# Autodesk Inventor assembly: Cabeza
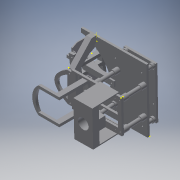
[picture p0: Inventor's stored thumbnail of the model, 180x180]
Saved by Autodesk Inventor 2017 SP1 (Build 210196100, 196)
## iProperties
Part Number: Cabeza
Material: Genérico
Document SubType Name: Assembly
Designer: Juan
Author: Juan
## Documents named in this file (13)
- C:\Users\Juan\Documents\Inventor\Cabeza_1\Cabeza.iam
- C:\Users\Juan\Documents\Inventor\Cabeza_1\BaseSuperior.ipt
- C:\Users\Juan\Documents\Inventor\Cabeza_1\Base.ipt
- C:\Users\Juan\Documents\Inventor\Cabeza_1\PosteLargo.ipt
- C:\Users\Juan\Documents\Inventor\Cabeza_1\PosteV.ipt
- C:\Users\Juan\Documents\Inventor\Cabeza_1\PosteCorto.ipt
- C:\Users\Juan\Documents\Inventor\Cabeza_1\BaseRB.ipt
- C:\Users\Juan\Documents\Inventor\Cabeza_1\SoporteCuello.ipt
- C:\Users\Juan\Documents\Inventor\Cabeza_1\PuenteMandibula.ipt
- C:\Users\Juan\Documents\Inventor\Cabeza_1\Mandibula.ipt
- C:\Users\Juan\Documents\Inventor\Cabeza_1\Puente.ipt
- C:\Users\Juan\Documents\Inventor\Cabeza_1\SoporteOjos.ipt
- C:\Users\Juan\Documents\Inventor\Cabeza_1\ojo.ipt
## Components (19 placed, 12 different names)
1. BaseSuperior:1 — Coincidencia:2, Coincidencia:3, Coincidencia:4, Coincidencia:5, Coincidencia:11, Coincidencia:14, Coincidencia:19
2. Base:1 — Coincidencia:7, Coincidencia:8, Coincidencia:9, Coincidencia:10, Coincidencia:12, Coincidencia:13, Coincidencia:15, Coincidencia:16, Coincidencia:17
3. PosteCorto:2 — Coincidencia:5
4. PosteCorto:3 — Coincidencia:4
5. PosteCorto:4 — Coincidencia:2
6. PosteCorto:5 — Coincidencia:3, Coincidencia:6
7. BaseRB:1 — Coincidencia:6
8. PosteLargo:2 — Coincidencia:9
9. PosteLargo:3 — Coincidencia:10, Coincidencia:14
10. PosteLargo:4 — Coincidencia:8
11. PosteLargo:5 — Coincidencia:7, Coincidencia:11
12. PosteV:1 — Coincidencia:12, Coincidencia:13
13. SoporteCuello:1 — Coincidencia:15, Coincidencia:16
14. PuenteMandibula:1 — Coincidencia:17, Coincidencia:18
15. Mandibula:1 — Coincidencia:18
16. Puente:1 — Coincidencia:19, Coincidencia:20
17. SoporteOjos:1 — Coincidencia:20, Coincidencia:21, Coincidencia:22
18. ojo:1 — Coincidencia:21
19. ojo:2 — Coincidencia:22
## Relationships (21: Mate 21)
- Coincidencia:2 [Mate]: BaseSuperior:1 ↔ PosteCorto:4
- Coincidencia:3 [Mate]: BaseSuperior:1 ↔ PosteCorto:5
- Coincidencia:4 [Mate]: BaseSuperior:1 ↔ PosteCorto:3
- Coincidencia:5 [Mate]: BaseSuperior:1 ↔ PosteCorto:2
- Coincidencia:6 [Mate]: PosteCorto:5 ↔ BaseRB:1
- Coincidencia:7 [Mate]: Base:1 ↔ PosteLargo:5
- Coincidencia:8 [Mate]: Base:1 ↔ PosteLargo:4
- Coincidencia:9 [Mate]: Base:1 ↔ PosteLargo:2
- Coincidencia:10 [Mate]: Base:1 ↔ PosteLargo:3
- Coincidencia:11 [Mate]: BaseSuperior:1 ↔ PosteLargo:5
- Coincidencia:12 [Mate]: Base:1 ↔ PosteV:1
- Coincidencia:13 [Mate]: Base:1 ↔ PosteV:1
- Coincidencia:14 [Mate]: BaseSuperior:1 ↔ PosteLargo:3
- Coincidencia:15 [Mate]: Base:1 ↔ SoporteCuello:1
- Coincidencia:16 [Mate]: Base:1 ↔ SoporteCuello:1
- Coincidencia:17 [Mate]: Base:1 ↔ PuenteMandibula:1
- Coincidencia:18 [Mate]: PuenteMandibula:1 ↔ Mandibula:1
- Coincidencia:19 [Mate]: BaseSuperior:1 ↔ Puente:1
- Coincidencia:20 [Mate]: Puente:1 ↔ SoporteOjos:1
- Coincidencia:21 [Mate]: SoporteOjos:1 ↔ ojo:1
- Coincidencia:22 [Mate]: SoporteOjos:1 ↔ ojo:2
